# Autodesk Inventor assembly: マブチRS380
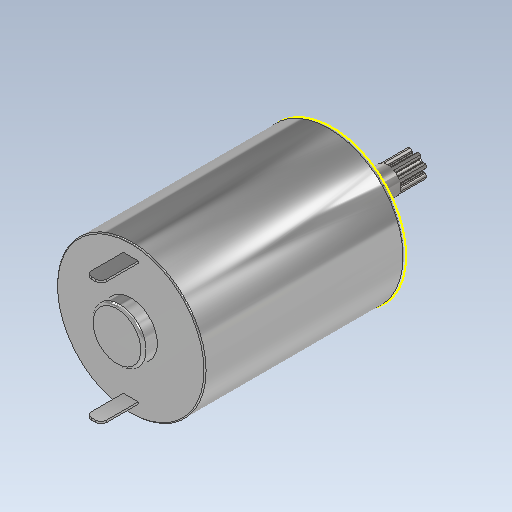
[picture p0: Inventor's stored thumbnail of the model, 512x512]
Saved by Autodesk Inventor 2020.2 (Build 242310000, 310)
## iProperties
Created: 2020-02-24
Part Number: マブチRS380
Document SubType Name: Assembly
Designer: aoyam
Mass: 81.3669 g
Surface Area: 52.7213 cm^2
Volume: 23.9008 cm^3
Density: 3.40436 g/cm^3
Author: aoyam
## Documents named in this file (3)
- C:\Users\aoyam\Desktop\SRDC_local\Inventor\二年機\Geminiβ\汎用部品\マブチRS380.iam
- C:\Users\aoyam\Desktop\SRDC_local\Inventor\二年機\Geminiβ\汎用部品\マブチRS-380PHピニオンz8.ipt
- C:\Users\aoyam\Desktop\SRDC_local\Inventor\二年機\Geminiβ\汎用部品\マブチRS-380本体.ipt
## Components (2 placed, 2 different names)
1. マブチRS-380PHピニオンz8:1 — 挿入:1
2. マブチRS-380本体:1 — 挿入:1
## Relationships (1: Insert 1)
- 挿入:1 [Insert]: マブチRS-380PHピニオンz8:1 ↔ マブチRS-380本体:1
